# Autodesk Inventor assembly: 200-20-ROCKER-CONNECTOR-ASM-01
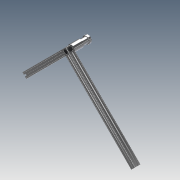
[picture p0: Inventor's stored thumbnail of the model, 180x180]
Saved by Autodesk Inventor 2018.2 (Build 222227000, 227)
## iProperties
Manager: feesmrt
Company: FRANC0R
Created: 2017-11-01
Part Number: 200-20-ROCKER-CONNECTOR-ASM-01
Material: Generisch
Document SubType Name: Assembly
Designer: feesmrt
Project: Rescue Robot
Cost Center: -
Description: Rocker Profile Connector
Engineer: feesmrt
Authority: feesmrt
Stock Number: 200-20-ROCKER-CONNECTOR-ASM-01
Author: feesmrt
Title: Rocker Profile Connector
Subject: Rescue Robot
Revision Number: 1
## Documents named in this file (9)
- D:\Programmierung\FRANC0R\CAD\02-Rocker-Bogie-Robot\200-ROCKER-BOGIE\200-20-ROCKER-CONNECTOR-ASM-01.iam
- D:\Programmierung\FRANC0R\CAD\02-Rocker-Bogie-Robot\200-ROCKER-BOGIE\200-20-ROCKER-CONNECTOR-01.ipt
- D:\Programmierung\FRANC0R\CAD\02-Rocker-Bogie-Robot\200-ROCKER-BOGIE\200-20-ROCKER-CONNECTOR-02.ipt
- D:\Programmierung\FRANC0R\CAD\02-Rocker-Bogie-Robot\900-COMPONENTS\900-40-SCREWS\900-40-SCREWS-ISO10642_M6x16.ipt
- D:\Programmierung\FRANC0R\CAD\02-Rocker-Bogie-Robot\900-COMPONENTS\900-50-PROFILES\90-50-PROFILES-QUAD-CONN-30x30.ipt
- D:\Programmierung\FRANC0R\CAD\02-Rocker-Bogie-Robot\900-COMPONENTS\900-50-PROFILES\90-50-PROFILES-30x30x300.ipt
- D:\Programmierung\FRANC0R\CAD\02-Rocker-Bogie-Robot\900-COMPONENTS\900-50-PROFILES\90-50-PROFILES-30x30x500.ipt
- D:\Programmierung\FRANC0R\CAD\02-Rocker-Bogie-Robot\900-COMPONENTS\900-40-SCREWS\900-40-SCREWS-ISO10642_M8x25.ipt
- D:\Programmierung\FRANC0R\CAD\02-Rocker-Bogie-Robot\900-COMPONENTS\900-50-PROFILES\90-50-PROFILES-QUAD-CONN-30x30-CAP.ipt
## Components (12 placed, 8 different names)
1. 200-20-ROCKER-CONNECTOR-01:1 — Passend:1, Passend:2, Passend:5, Passend:6, Passend:7, Passend:12
2. 200-20-ROCKER-CONNECTOR-02:1 — Passend:1, Passend:2, Passend:4, Fluchtend:1
3. 900-40-SCREWS-ISO10642_M6x16:1 — Passend:4, Fluchtend:1
4. 90-50-PROFILES-QUAD-CONN-30x30:1 — Passend:5, Passend:6, Passend:7, Passend:8, Fluchtend:2, Passend:9, Passend:10, Fluchtend:3, Passend:11, Fluchtend:4, Fluchtend:5, Passend:14, Fluchtend:6, Passend:15, Passend:16, Passend:17, Passend:18, Passend:19, Passend:20
5. 90-50-PROFILES-30x30x300:1 — Passend:8, Fluchtend:2, Passend:9, Passend:13
6. 90-50-PROFILES-30x30x500:1 — Passend:10, Fluchtend:3, Passend:11
7. 900-40-SCREWS-ISO10642_M8x25:1 — Passend:12, Fluchtend:4
8. 900-40-SCREWS-ISO10642_M8x25:2 — Passend:13, Fluchtend:5
9. 900-40-SCREWS-ISO10642_M8x25:3 — Passend:14, Fluchtend:6
10. 90-50-PROFILES-QUAD-CONN-30x30-CAP:2 — Passend:17, Passend:18
11. 90-50-PROFILES-QUAD-CONN-30x30-CAP:3 — Passend:15, Passend:16
12. 90-50-PROFILES-QUAD-CONN-30x30-CAP:4 — Passend:19, Passend:20
## Relationships (25: Mate 19, Flush 6)
- Passend:1 [Mate]: 200-20-ROCKER-CONNECTOR-01:1 ↔ 200-20-ROCKER-CONNECTOR-02:1
- Passend:2 [Mate]: 200-20-ROCKER-CONNECTOR-01:1 ↔ 200-20-ROCKER-CONNECTOR-02:1
- Passend:4 [Mate]: 200-20-ROCKER-CONNECTOR-02:1 ↔ 900-40-SCREWS-ISO10642_M6x16:1
- Fluchtend:1 [Flush]: 200-20-ROCKER-CONNECTOR-02:1 ↔ 900-40-SCREWS-ISO10642_M6x16:1
- Passend:5 [Mate]: 200-20-ROCKER-CONNECTOR-01:1 ↔ 90-50-PROFILES-QUAD-CONN-30x30:1
- Passend:6 [Mate]: 200-20-ROCKER-CONNECTOR-01:1 ↔ 90-50-PROFILES-QUAD-CONN-30x30:1
- Passend:7 [Mate]: 200-20-ROCKER-CONNECTOR-01:1 ↔ 90-50-PROFILES-QUAD-CONN-30x30:1
- Passend:8 [Mate]: 90-50-PROFILES-QUAD-CONN-30x30:1 ↔ 90-50-PROFILES-30x30x300:1
- Fluchtend:2 [Flush]: 90-50-PROFILES-QUAD-CONN-30x30:1 ↔ 90-50-PROFILES-30x30x300:1
- Passend:9 [Mate]: 90-50-PROFILES-QUAD-CONN-30x30:1 ↔ 90-50-PROFILES-30x30x300:1
- Passend:10 [Mate]: 90-50-PROFILES-QUAD-CONN-30x30:1 ↔ 90-50-PROFILES-30x30x500:1
- Fluchtend:3 [Flush]: 90-50-PROFILES-QUAD-CONN-30x30:1 ↔ 90-50-PROFILES-30x30x500:1
- Passend:11 [Mate]: 90-50-PROFILES-QUAD-CONN-30x30:1 ↔ 90-50-PROFILES-30x30x500:1
- Passend:12 [Mate]: 200-20-ROCKER-CONNECTOR-01:1 ↔ 900-40-SCREWS-ISO10642_M8x25:1
- Fluchtend:4 [Flush]: 90-50-PROFILES-QUAD-CONN-30x30:1 ↔ 900-40-SCREWS-ISO10642_M8x25:1
- Passend:13 [Mate]: 90-50-PROFILES-30x30x300:1 ↔ 900-40-SCREWS-ISO10642_M8x25:2
- Fluchtend:5 [Flush]: 90-50-PROFILES-QUAD-CONN-30x30:1 ↔ 900-40-SCREWS-ISO10642_M8x25:2
- Passend:14 [Mate]: 90-50-PROFILES-QUAD-CONN-30x30:1 ↔ 900-40-SCREWS-ISO10642_M8x25:3
- Fluchtend:6 [Flush]: 90-50-PROFILES-QUAD-CONN-30x30:1 ↔ 900-40-SCREWS-ISO10642_M8x25:3
- Passend:15 [Mate]: 90-50-PROFILES-QUAD-CONN-30x30:1 ↔ 90-50-PROFILES-QUAD-CONN-30x30-CAP:3
- Passend:16 [Mate]: 90-50-PROFILES-QUAD-CONN-30x30:1 ↔ 90-50-PROFILES-QUAD-CONN-30x30-CAP:3
- Passend:17 [Mate]: 90-50-PROFILES-QUAD-CONN-30x30:1 ↔ 90-50-PROFILES-QUAD-CONN-30x30-CAP:2
- Passend:18 [Mate]: 90-50-PROFILES-QUAD-CONN-30x30:1 ↔ 90-50-PROFILES-QUAD-CONN-30x30-CAP:2
- Passend:19 [Mate]: 90-50-PROFILES-QUAD-CONN-30x30:1 ↔ 90-50-PROFILES-QUAD-CONN-30x30-CAP:4
- Passend:20 [Mate]: 90-50-PROFILES-QUAD-CONN-30x30:1 ↔ 90-50-PROFILES-QUAD-CONN-30x30-CAP:4
